# Autodesk Inventor assembly: Conjunto polea motor 2
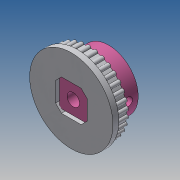
[picture p0: Inventor's stored thumbnail of the model, 180x180]
Saved by Autodesk Inventor 2017 (Build 210142000, 142)
## iProperties
Part Number: Conjunto polea motor 2
Material: Genérico
Document SubType Name: Assembly
Designer: FABLAB
Author: FABLAB
## Documents named in this file (3)
- C:\Users\Leo\Documents\GitHub\actor-re-actor\models\inventor-caja\partes transmision\Conjunto polea motor 2.iam
- C:\Users\Leo\Documents\GitHub\actor-re-actor\models\inventor-caja\partes transmision\dado polea.ipt
- C:\Users\Leo\Documents\GitHub\actor-re-actor\models\inventor-caja\partes transmision\engrane correa dado-motor 2.ipt
## Components (2 placed, 2 different names)
1. dado polea:1 — Nivelación:1
2. engrane correa dado-motor 2:1 — Nivelación:1, Coincidencia:1, Coincidencia:2
## Relationships (3: Mate 2, Flush 1)
- Nivelación:1 [Flush]: dado polea:1 ↔ engrane correa dado-motor 2:1
- Coincidencia:1 [Mate]: engrane correa dado-motor 2:1
- Coincidencia:2 [Mate]: engrane correa dado-motor 2:1
